# Autodesk Inventor assembly: M - hook block V2
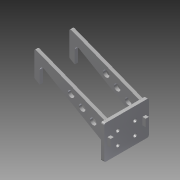
[picture p0: Inventor's stored thumbnail of the model, 180x180]
Saved by Autodesk Inventor 2013 (Build 170138000, 138)
## iProperties
Created: 2013-01-27
Part Number: M - hook block V2
Document SubType Name: Assembly
Designer: Arpan
Mass: 1657.38 g
Surface Area: 867.213 cm^2
Volume: 211.132 cm^3
Density: 7.85 g/cm^3
Author: Arpan
## Documents named in this file (3)
- C:\Users\Moses\Documents\GitHub\frc2013CAD\M-Climber\M - hook block V2.iam
- C:\Users\Moses\Documents\GitHub\frc2013CAD\Cimber actual\hook faceplate.ipt
- C:\Users\Moses\Documents\GitHub\frc2013CAD\Cimber actual\hook.ipt
## Components (3 placed, 2 different names)
1. hook faceplate:1 — Mate:7, Mate:8, Mate:9, Mate:10, Mate:11, Mate:12
2. hook:1 — Mate:10, Mate:11, Mate:12
3. hook:2 — Mate:7, Mate:8, Mate:9
## Relationships (6: Mate 6)
- Mate:7: hook faceplate:1 ↔ hook:2
- Mate:8: hook faceplate:1 ↔ hook:2
- Mate:9: hook faceplate:1 ↔ hook:2
- Mate:10: hook faceplate:1 ↔ hook:1
- Mate:11: hook faceplate:1 ↔ hook:1
- Mate:12: hook faceplate:1 ↔ hook:1
